# Autodesk Inventor assembly: controller
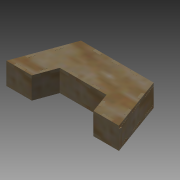
[picture p0: Inventor's stored thumbnail of the model, 180x180]
Saved by Autodesk Inventor 2015 (Build 190159000, 159)
## iProperties
Created: 2015-10-06
Part Number: controller
Document SubType Name: Assembly
Designer: Haukur
Author: Haukur
## Documents named in this file (7)
- C:\haukur\skoli\5.onn\Mech\inventor\controller\controller.iam
- C:\haukur\skoli\5.onn\Mech\inventor\controller\back.ipt
- C:\haukur\skoli\5.onn\Mech\inventor\controller\front(vga).ipt
- C:\haukur\skoli\5.onn\Mech\inventor\controller\hlid.ipt
- C:\haukur\skoli\5.onn\Mech\inventor\controller\stubbur.ipt
- C:\haukur\skoli\5.onn\Mech\inventor\controller\innanverdurstubbur.ipt
- C:\haukur\skoli\5.onn\Mech\inventor\controller\front(magi).ipt
## Components (10 placed, 6 different names)
1. back:1 — Mate:1, Mate:2, Mate:3, Mate:4, Mate:5, Mate:6, Mate:7, Mate:8, Mate:9, Mate:10, Mate:11, Mate:12, Mate:13, Mate:14, Mate:15, Mate:16, Mate:17, Mate:18, Mate:19, Mate:20, Mate:21, Mate:22, Mate:23, Mate:24
2. front(vga):1 — Mate:1, Mate:2, Mate:3, Mate:26, Mate:27
3. hlid:1 — Mate:4, Mate:5, Mate:6
4. hlid:2 — Mate:7, Mate:8, Mate:9
5. stubbur:1 — Mate:13, Mate:14, Mate:15
6. stubbur:2 — Mate:10, Mate:11, Mate:12
7. innanverdurstubbur:1 — Mate:16, Mate:17, Mate:18
8. innanverdurstubbur:2 — Mate:19, Mate:20, Mate:21
9. front(magi):1 — Mate:22, Mate:23, Mate:24, Mate:25
10. back:2 — Mate:25, Mate:26, Mate:27
## Relationships (27: Mate 27)
- Mate:1: back:1 ↔ front(vga):1
- Mate:2: back:1 ↔ front(vga):1
- Mate:3: back:1 ↔ front(vga):1
- Mate:4: back:1 ↔ hlid:1
- Mate:5: back:1 ↔ hlid:1
- Mate:6: back:1 ↔ hlid:1
- Mate:7: back:1 ↔ hlid:2
- Mate:8: back:1 ↔ hlid:2
- Mate:9: back:1 ↔ hlid:2
- Mate:10: back:1 ↔ stubbur:2
- Mate:11: back:1 ↔ stubbur:2
- Mate:12: back:1 ↔ stubbur:2
- Mate:13: back:1 ↔ stubbur:1
- Mate:14: back:1 ↔ stubbur:1
- Mate:15: back:1 ↔ stubbur:1
- Mate:16: back:1 ↔ innanverdurstubbur:1
- Mate:17: back:1 ↔ innanverdurstubbur:1
- Mate:18: back:1 ↔ innanverdurstubbur:1
- Mate:19: back:1 ↔ innanverdurstubbur:2
- Mate:20: back:1 ↔ innanverdurstubbur:2
- Mate:21: back:1 ↔ innanverdurstubbur:2
- Mate:22: back:1 ↔ front(magi):1
- Mate:23: back:1 ↔ front(magi):1
- Mate:24: back:1 ↔ front(magi):1
- Mate:25: front(magi):1 ↔ back:2
- Mate:26: front(vga):1 ↔ back:2
- Mate:27: front(vga):1 ↔ back:2
